# Autodesk Inventor assembly: Microlab_Electrical_CAD
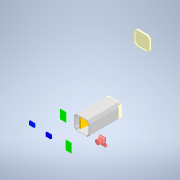
[picture p0: Inventor's stored thumbnail of the model, 180x180]
Saved by Autodesk Inventor 2022 (Build 260153000, 153)
## iProperties
Created: 2021-09-30
Part Number: Microlab_Electrical_CAD
Document SubType Name: Assembly
Designer: iss
Author: iss
## Documents named in this file (9)
- C:\Users\ISS\Downloads\Microlab_Electrical_CAD (1).iam
- C:\Users\ISS\Downloads\TPA6021A4EVM.ipt
- C:\Users\ISS\Downloads\AD9833Teyleten.ipt
- C:\Users\ISS\Downloads\OneDrive_1_9-28-2021\MicroLab_Center_Shell.ipt
- C:\Users\ISS\Downloads\APS3008S-R.ipt
- C:\Users\ISS\Downloads\OneDrive_1_9-28-2021\C329-SPI.ipt
- C:\Users\ISS\Downloads\OneDrive_1_9-28-2021\MicroLab_Rear_Cover.ipt
- C:\Users\ISS\Downloads\OneDrive_1_9-28-2021\MicroLab_Front_Cover.ipt
- C:\Users\ISS\Downloads\OneDrive_1_9-28-2021\MicroLab_PCB_002.ipt
## Components (10 placed, 8 different names)
1. TPA6021A4EVM:1
2. AD9833Teyleten:1
3. MicroLab_Center_Shell:1 — Mate:4
4. AD9833Teyleten:2
5. APS3008S-R:1
6. APS3008S-R:2
7. C329-SPI:1
8. MicroLab_Rear_Cover:1 — Mate:1, Mate:2, Mate:3, Mate:4
9. MicroLab_Front_Cover:1
10. MicroLab_PCB_002:1 — Mate:1, Mate:2, Mate:3
## Relationships (4: Mate 4)
- Mate:1: MicroLab_Rear_Cover:1 ↔ MicroLab_PCB_002:1
- Mate:2: MicroLab_Rear_Cover:1 ↔ MicroLab_PCB_002:1
- Mate:3: MicroLab_Rear_Cover:1 ↔ MicroLab_PCB_002:1
- Mate:4: MicroLab_Center_Shell:1 ↔ MicroLab_Rear_Cover:1
